# Autodesk Inventor assembly: Сборка1
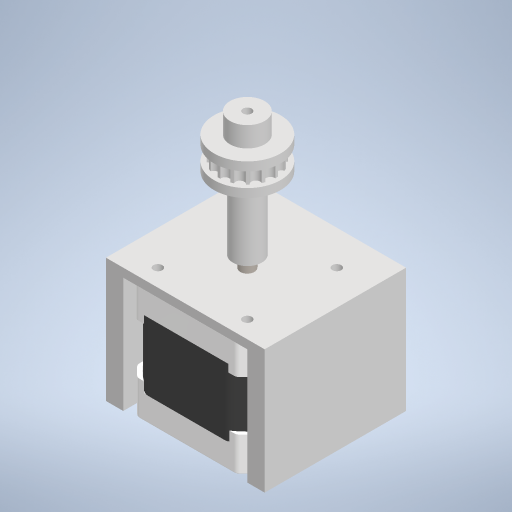
[picture p0: Inventor's stored thumbnail of the model, 512x512]
Saved by Autodesk Inventor 2023 (Build 270158000, 158)
## iProperties
Created: 2023-04-09
Part Number: Сборка1
Document SubType Name: Assembly
Designer: deryu
Author: deryu
## Documents named in this file (6)
- C:\Users\deryu\OneDrive\Рабочий стол\Лампа\Управление гардиной\3д модель\Сборка1.iam
- C:\Users\deryu\OneDrive\Рабочий стол\Лампа\Управление гардиной\3д модель\вращалка.ipt
- C:\Users\deryu\OneDrive\Рабочий стол\Лампа\Управление гардиной\3д модель\motor-nema-17-40mm-1.snapshot.1\NEMA17\Inventor\17HM15-0904S.iam
- C:\Users\deryu\OneDrive\Рабочий стол\Лампа\Управление гардиной\3д модель\передача момента.ipt
- C:\Users\deryu\OneDrive\Рабочий стол\Лампа\Управление гардиной\3д модель\крышка для втулки.ipt
- C:\Users\deryu\OneDrive\Рабочий стол\Лампа\Управление гардиной\3д модель\Держатель.ipt
## Components (5 placed, 5 different names)
1. вращалка:1 — Совмещение:5, Совмещение:7, Совмещение:8, Совмещение:9
2. 17HM15-0904S:1 [sub-assembly] — Совмещение:1, Совмещение:2, Совмещение:3, Совмещение:4, Совмещение:6, Заподлицо:1
3. передача момента:1 — Совмещение:1, Совмещение:3, Совмещение:5, Совмещение:6, Совмещение:7
4. крышка для втулки:1 — Совмещение:8, Совмещение:9
5. Держатель:1 — Заподлицо:1
## Relationships (10: Mate 9, Flush 1)
- Совмещение:1 [Mate]: 17HM15-0904S:1 ↔ передача момента:1
- Совмещение:2 [Mate]: 17HM15-0904S:1
- Совмещение:3 [Mate]: 17HM15-0904S:1 ↔ передача момента:1
- Совмещение:4 [Mate]: 17HM15-0904S:1
- Совмещение:5 [Mate]: вращалка:1 ↔ передача момента:1
- Совмещение:6 [Mate]: 17HM15-0904S:1 ↔ передача момента:1
- Совмещение:7 [Mate]: вращалка:1 ↔ передача момента:1
- Совмещение:8 [Mate]: вращалка:1 ↔ крышка для втулки:1
- Совмещение:9 [Mate]: вращалка:1 ↔ крышка для втулки:1
- Заподлицо:1 [Flush]: 17HM15-0904S:1 ↔ Держатель:1
